# Autodesk Inventor assembly: SCREEN HOLDER 3P
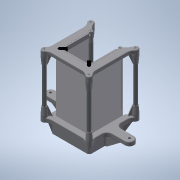
[picture p0: Inventor's stored thumbnail of the model, 180x180]
Saved by Autodesk Inventor 2020.3 (Build 243373000, 373)
## iProperties
RuleStatus: InUse
AfterDocSave0: file://Part Number Cleaner
Created: 2023-03-02
Catalog Web Link: https://www.janelia.org/
Vendor: HHMI: JRC - jET
Document SubType Name: Assembly
Designer: jalala
DESIGN DEPARTMENT: HHMI: JRC - jET
ALTERED ITEM PART NUMBER: N/A
ALTERED ITEM VENDOR: N/A
ALTERED ITEM DESCRIPTION: N/A
PART NUMBER - LEGACY: Standard
Author: jalala
Revision Number: 0
## Documents named in this file (13)
- C:\_WORKSPACE\DATA\PROJECTS\_PROJECTS BY LAB\VIVEK (LAB)\4 PROJECTOR FLY VR RIG\3 PROJECTOR SCREEN ASSEMBLY\SCREEN HOLDER 3P.iam
- C:\_WORKSPACE\DATA\PROJECTS\_PROJECTS BY LAB\VIVEK (LAB)\4 PROJECTOR FLY VR RIG\3 PROJECTOR SCREEN ASSEMBLY\WIDE SCREEN HOLDER 3P.ipt
- C:\_WORKSPACE\DATA\PROJECTS\_PROJECTS BY LAB\VIVEK (LAB)\4 PROJECTOR FLY VR RIG\3 PROJECTOR SCREEN ASSEMBLY\WIDE SCREEN HOLDER 3P_MIR.ipt
- C:\_WORKSPACE\DATA\PROJECTS\_PROJECTS BY LAB\VIVEK (LAB)\4 PROJECTOR FLY VR RIG\3 PROJECTOR SCREEN ASSEMBLY\TOP SCREEN SUPPORT 3P FRAME.ipt
- C:\_WORKSPACE\DATA\PROJECTS\_PROJECTS BY LAB\VIVEK (LAB)\4 PROJECTOR FLY VR RIG\3 PROJECTOR SCREEN ASSEMBLY\BOTTOM SCREEN SUPPORT 3P.ipt
- C:\_WORKSPACE\DATA\PROJECTS\_PROJECTS BY LAB\VIVEK (LAB)\4 PROJECTOR FLY VR RIG\3 PROJECTOR SCREEN ASSEMBLY\SCREEN ASSEMBLY GUIDE 3P.ipt
- C:\_WORKSPACE\DATA\PROJECTS\_PROJECTS BY LAB\VIVEK (LAB)\4 PROJECTOR FLY VR RIG\3 PROJECTOR SCREEN ASSEMBLY\SCREEN ASSEMBLY GUIDE 3P_MIR.ipt
- C:\_WORKSPACE\DATA\PROJECTS\_PROJECTS BY LAB\VIVEK (LAB)\4 PROJECTOR FLY VR RIG\3 PROJECTOR SCREEN ASSEMBLY\SCREEN 3P.ipt
- C:\_WORKSPACE\DATA\COMMON\Thorlabs\MS3R.ipt
- C:\_WORKSPACE\DATA\PROJECTS\_PROJECTS BY LAB\VIVEK (LAB)\4 PROJECTOR FLY VR RIG\91500A120_316 Stainless Steel Phillips Flat Head Screws.ipt
- C:\_WORKSPACE\DATA\PROJECTS\_PROJECTS BY LAB\VIVEK (LAB)\4 PROJECTOR FLY VR RIG\91500A308_316 Stainless Steel Phillips Flat Head Screws.ipt
- C:\_WORKSPACE\DATA\PROJECTS\_PROJECTS BY LAB\VIVEK (LAB)\4 PROJECTOR FLY VR RIG\91500A120_316 Stainless Steel Phillips Flat Head Screws_MIR.ipt
- C:\_WORKSPACE\DATA\PROJECTS\_PROJECTS BY LAB\VIVEK (LAB)\4 PROJECTOR FLY VR RIG\3 PROJECTOR SCREEN ASSEMBLY\CENTERING JIG 3P.ipt
## Components (30 placed, 12 different names)
1. WIDE SCREEN HOLDER 3P:1 — Flush:1, Flush:3, Mate:2, Angle:1, Flush:5
2. WIDE SCREEN HOLDER 3P_MIR:1 — Mate:1, Flush:2, Rigid:1, Rigid:2
3. TOP SCREEN SUPPORT 3P FRAME:1 — Flush:2, Rotational:1, Rotational:2, Rotational:3, Rotational:4, Flush:6, Rigid:3, Rigid:4, Rigid:5, Rigid:6
4. BOTTOM SCREEN SUPPORT 3P:1 — Flush:3, Flush:7
5. SCREEN ASSEMBLY GUIDE 3P:1 — Flush:4
6. SCREEN ASSEMBLY GUIDE 3P_MIR:1 — Mate:3
7. SCREEN 3P:1 — Flush:5
8. MS3R:1 — Rigid:1
9. MS3R:2 — Rigid:2
10. 91500A120_316 Stainless Steel Phillips Flat Head Screws:1 — Rotational:1
11. 91500A120_316 Stainless Steel Phillips Flat Head Screws:2 — Rotational:2
12. 91500A120_316 Stainless Steel Phillips Flat Head Screws:3 — Rotational:3
13. 91500A120_316 Stainless Steel Phillips Flat Head Screws:4 — Rotational:4
14. 91500A120_316 Stainless Steel Phillips Flat Head Screws_MIR:1
15. 91500A120_316 Stainless Steel Phillips Flat Head Screws_MIR:2
16. 91500A120_316 Stainless Steel Phillips Flat Head Screws_MIR:3
17. 91500A120_316 Stainless Steel Phillips Flat Head Screws_MIR:4 — Flush:7
18. CENTERING JIG 3P:1
19. MS3R:3 — Rigid:4
20. MS3R:4 — Rigid:3
21. 91500A308_316 Stainless Steel Phillips Flat Head Screws:1 — Rigid:5
22. 91500A308_316 Stainless Steel Phillips Flat Head Screws:2 — Rigid:6
23. 91500A308_316 Stainless Steel Phillips Flat Head Screws:3
24. 91500A308_316 Stainless Steel Phillips Flat Head Screws:4
25. 91500A308_316 Stainless Steel Phillips Flat Head Screws:5
26. 91500A308_316 Stainless Steel Phillips Flat Head Screws:6
27. 91500A308_316 Stainless Steel Phillips Flat Head Screws:7
28. 91500A308_316 Stainless Steel Phillips Flat Head Screws:8
29. MS3R:5
30. MS3R:6
## Relationships (21: Flush 7, WeldJoint 6, RevoluteJoint 4, Mate 3, Angle 1)
- Flush:1 (47.625 mm): WIDE SCREEN HOLDER 3P:1
- Mate:1 (47.625 mm): WIDE SCREEN HOLDER 3P_MIR:1
- Flush:2: WIDE SCREEN HOLDER 3P_MIR:1 ↔ TOP SCREEN SUPPORT 3P FRAME:1
- Flush:3: WIDE SCREEN HOLDER 3P:1 ↔ BOTTOM SCREEN SUPPORT 3P:1
- Mate:2: WIDE SCREEN HOLDER 3P:1
- Angle:1 (45 deg): WIDE SCREEN HOLDER 3P:1
- Flush:4: SCREEN ASSEMBLY GUIDE 3P:1
- Mate:3: SCREEN ASSEMBLY GUIDE 3P_MIR:1
- Flush:5: WIDE SCREEN HOLDER 3P:1 ↔ SCREEN 3P:1
- Rigid:1 [WeldJoint]: WIDE SCREEN HOLDER 3P_MIR:1 ↔ MS3R:1
- Rigid:2 [WeldJoint]: WIDE SCREEN HOLDER 3P_MIR:1 ↔ MS3R:2
- Rotational:1 [RevoluteJoint]: TOP SCREEN SUPPORT 3P FRAME:1 ↔ 91500A120_316 Stainless Steel Phillips Flat Head Screws:1
- Rotational:2 [RevoluteJoint]: TOP SCREEN SUPPORT 3P FRAME:1 ↔ 91500A120_316 Stainless Steel Phillips Flat Head Screws:2
- Rotational:3 [RevoluteJoint]: TOP SCREEN SUPPORT 3P FRAME:1 ↔ 91500A120_316 Stainless Steel Phillips Flat Head Screws:3
- Rotational:4 [RevoluteJoint]: TOP SCREEN SUPPORT 3P FRAME:1 ↔ 91500A120_316 Stainless Steel Phillips Flat Head Screws:4
- Flush:6 (-54.61 mm): TOP SCREEN SUPPORT 3P FRAME:1
- Rigid:3 [WeldJoint]: TOP SCREEN SUPPORT 3P FRAME:1 ↔ MS3R:4
- Rigid:4 [WeldJoint]: TOP SCREEN SUPPORT 3P FRAME:1 ↔ MS3R:3
- Rigid:5 [WeldJoint]: TOP SCREEN SUPPORT 3P FRAME:1 ↔ 91500A308_316 Stainless Steel Phillips Flat Head Screws:1
- Rigid:6 [WeldJoint]: TOP SCREEN SUPPORT 3P FRAME:1 ↔ 91500A308_316 Stainless Steel Phillips Flat Head Screws:2
- Flush:7: BOTTOM SCREEN SUPPORT 3P:1 ↔ 91500A120_316 Stainless Steel Phillips Flat Head Screws_MIR:4
